# Autodesk Inventor assembly: Assembly
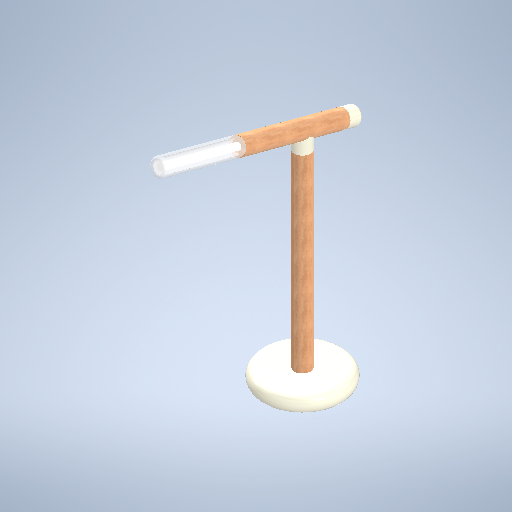
[picture p0: Inventor's stored thumbnail of the model, 512x512]
Saved by Autodesk Inventor 2025.3 (Build 293356000, 356)
## iProperties
Created: 2026-01-15
Part Number: Assembly
Document SubType Name: Assembly
Designer: Balint
Author: Balint
## Documents named in this file (9)
- C:\Users\Balint\3D\Dlamp\Assembly.iam
- C:\Users\Balint\3D\Dlamp\Base.ipt
- C:\Users\Balint\3D\Dlamp\Base_Cover.ipt
- C:\Users\Balint\3D\Dlamp\Dowel2.ipt
- C:\Users\Balint\3D\Dlamp\Joint.ipt
- C:\Users\Balint\3D\Dlamp\Dowel1.ipt
- C:\Users\Balint\3D\Dlamp\Brightness.ipt
- C:\Users\Balint\3D\Dlamp\LightPole.ipt
- C:\Users\Balint\3D\Dlamp\Diffueser.ipt
## Components (8 placed, 8 different names)
1. Base:1 — Mate:1, Mate:2, Mate:3, Mate:4, Mate:5, Mate:6
2. Base_Cover:1 — Mate:1, Mate:2, Mate:3
3. Dowel2:1 — Mate:4, Mate:5, Mate:6, Mate:7, Mate:8, Mate:9
4. Joint:1 — Mate:7, Mate:8, Mate:9, Mate:10, Tangent:1
5. Dowel1:1 — Mate:10, Tangent:1, Mate:11, Mate:12, Mate:13, Mate:14, Mate:16
6. Brightness:1 — Mate:11, Mate:12
7. LightPole:1 — Mate:13, Mate:14, Mate:15
8. Diffueser:1 — Mate:15, Mate:16
## Relationships (17: Mate 16, Tangent 1)
- Mate:1: Base:1 ↔ Base_Cover:1
- Mate:2: Base:1 ↔ Base_Cover:1
- Mate:3: Base:1 ↔ Base_Cover:1
- Mate:4: Base:1 ↔ Dowel2:1
- Mate:5: Base:1 ↔ Dowel2:1
- Mate:6: Base:1 ↔ Dowel2:1
- Mate:7: Dowel2:1 ↔ Joint:1
- Mate:8: Dowel2:1 ↔ Joint:1
- Mate:9: Dowel2:1 ↔ Joint:1
- Mate:10: Joint:1 ↔ Dowel1:1
- Tangent:1: Joint:1 ↔ Dowel1:1
- Mate:11: Dowel1:1 ↔ Brightness:1
- Mate:12 (0.5 mm): Dowel1:1 ↔ Brightness:1
- Mate:13: Dowel1:1 ↔ LightPole:1
- Mate:14: Dowel1:1 ↔ LightPole:1
- Mate:15: LightPole:1 ↔ Diffueser:1
- Mate:16: Dowel1:1 ↔ Diffueser:1
